# Autodesk Inventor assembly: PHolder
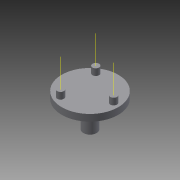
[picture p0: Inventor's stored thumbnail of the model, 180x180]
Saved by Autodesk Inventor 2014 (Build 180170000, 170)
## iProperties
Created: 2013-05-25
Part Number: PHolder
Document SubType Name: Assembly
Designer: Felix
Author: Felix
## Documents named in this file (3)
- C:\Users\Felix\Desktop\Beep\Hardware\Z132053\PHolderEnd.iam
- C:\Users\Felix\Desktop\PSteg.ipt
- C:\Users\Felix\Desktop\Beep\Hardware\Z132053\WelleOut.ipt
## Components (2 placed, 2 different names)
1. PSteg:1 — Mate:2, Mate:4, Flush:1
2. WelleOut:1 — Flush:1, Mate:5
## Relationships (4: Mate 3, Flush 1)
- Mate:2: PSteg:1
- Mate:4: PSteg:1
- Flush:1: PSteg:1 ↔ WelleOut:1
- Mate:5: WelleOut:1
